# Autodesk Inventor assembly: y-carriage
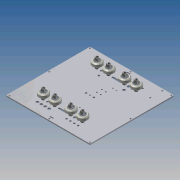
[picture p0: Inventor's stored thumbnail of the model, 180x180]
Saved by Autodesk Inventor 2015 (Build 190159000, 159)
## iProperties
Created: 2015-10-04
Part Number: y-carriage
Document SubType Name: Assembly
Designer: Solomon
Author: Solomon
## Documents named in this file (3)
- C:\Users\Solomon\Documents\Inventor\Omni 1\y-carriage.iam
- C:\Users\Solomon\Documents\Inventor\Omni 1\V Slot Part Files\V Slot Plates\Universal Build Pate.ipt
- C:\Users\Solomon\Documents\Inventor\Omni 1\V Slot Part Files\assembledwheel.iam
## Components (9 placed, 2 different names)
1. Universal Build Pate:1 — Mate:1, Mate:2, Mate:3, Mate:4, Angle:1, Angle:2, Angle:3, Angle:4, Angle:5, Angle:6, Angle:7, Angle:8, Mate:5, Mate:6, Mate:7, Mate:8, Angle:9, Angle:10, Angle:11, Angle:12, Angle:13
2. assembledwheel:1 [sub-assembly] — Mate:1, Angle:3, Angle:8
3. assembledwheel:2 [sub-assembly] — Mate:2, Angle:2, Angle:5
4. assembledwheel:3 [sub-assembly] — Mate:3, Angle:1, Angle:6, Angle:9
5. assembledwheel:4 [sub-assembly] — Mate:4, Angle:4, Angle:7
6. assembledwheel:5 [sub-assembly] — Mate:5, Angle:12
7. assembledwheel:6 [sub-assembly] — Mate:6, Angle:13
8. assembledwheel:7 [sub-assembly] — Mate:8, Angle:11
9. assembledwheel:8 [sub-assembly] — Mate:7, Angle:10
## Relationships (21: Angle 13, Mate 8)
- Mate:1: Universal Build Pate:1 ↔ assembledwheel:1
- Mate:2: Universal Build Pate:1 ↔ assembledwheel:2
- Mate:3: Universal Build Pate:1 ↔ assembledwheel:3
- Mate:4: Universal Build Pate:1 ↔ assembledwheel:4
- Angle:1 (0 deg): Universal Build Pate:1 ↔ assembledwheel:3
- Angle:2 (0 deg): Universal Build Pate:1 ↔ assembledwheel:2
- Angle:3 (0 deg): Universal Build Pate:1 ↔ assembledwheel:1
- Angle:4 (0 deg): Universal Build Pate:1 ↔ assembledwheel:4
- Angle:5 (0 deg): Universal Build Pate:1 ↔ assembledwheel:2
- Angle:6 (0 deg): Universal Build Pate:1 ↔ assembledwheel:3
- Angle:7 (0 deg): Universal Build Pate:1 ↔ assembledwheel:4
- Angle:8 (0 deg): Universal Build Pate:1 ↔ assembledwheel:1
- Mate:5: Universal Build Pate:1 ↔ assembledwheel:5
- Mate:6: Universal Build Pate:1 ↔ assembledwheel:6
- Mate:7: Universal Build Pate:1 ↔ assembledwheel:8
- Mate:8: Universal Build Pate:1 ↔ assembledwheel:7
- Angle:9 (0 deg): Universal Build Pate:1 ↔ assembledwheel:3
- Angle:10 (0 deg): Universal Build Pate:1 ↔ assembledwheel:8
- Angle:11 (0 deg): Universal Build Pate:1 ↔ assembledwheel:7
- Angle:12 (0 deg): Universal Build Pate:1 ↔ assembledwheel:5
- Angle:13 (0 deg): Universal Build Pate:1 ↔ assembledwheel:6
